# Autodesk Inventor assembly: EnsambleBaseMotor
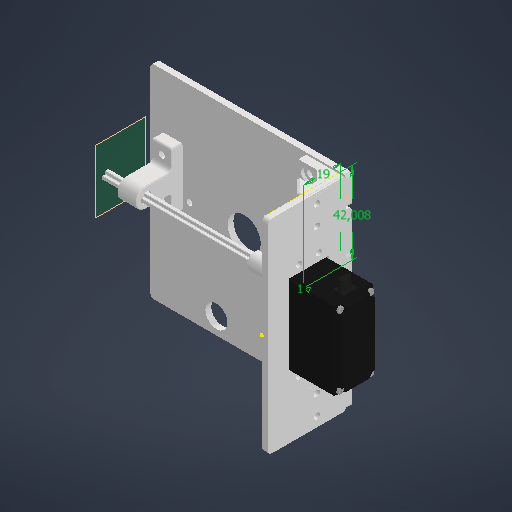
[picture p0: Inventor's stored thumbnail of the model, 512x512]
Saved by Autodesk Inventor 2026.3 (Build 303398000, 398)
## iProperties
Created: 2026-04-28
Part Number: EnsambleBaseMotor
Document SubType Name: Assembly
Designer: Jose Carlos
Author: Jose Carlos
## Documents named in this file (8)
- C:\Users\Caro\JoseCarlos\TEC\TFG\Inventor\PiezasSTD\EnsambleMotor\EnsambleBaseMotor.iam
- C:\Users\Caro\JoseCarlos\TEC\TFG\Inventor\PiezasSTD\EnsambleMotor\BaseMotoJose.ipt
- C:\Users\Caro\JoseCarlos\TEC\TFG\Inventor\PiezasSTD\EnsambleMotor\ParedEnsambleMotor.ipt
- C:\Users\Caro\JoseCarlos\TEC\TFG\Inventor\PiezasSTD\T.ipt
- C:\Users\Caro\JoseCarlos\TEC\TFG\Inventor\PiezasSTD\EnsambleMotor\AcopleMotor.ipt
- C:\Users\Caro\JoseCarlos\TEC\TFG\Inventor\PiezasSTD\EnsambleMotor\EjeDelMotor.ipt
- C:\Users\Caro\JoseCarlos\TEC\TFG\Inventor\Elementos\mg995-servo-motor-metal-gear-high-torque-standard-size-1.snapshot.1\MG995.ipt
- C:\Users\Caro\JoseCarlos\TEC\TFG\Inventor\PiezasSTD\EnsambleMotor\SoporteEjeMotor.ipt
## Components (12 placed, 7 different names)
1. BaseMotoJose:1 — Nivelación:1, Coincidencia:1, Coincidencia:4, Nivelación:3, Coincidencia:7, Nivelación:4, Coincidencia:9, Nivelación:5, Coincidencia:10, Ángulo:6, Nivelación:6, Ángulo:7, Coincidencia:26, Coincidencia:27, Coincidencia:28, Coincidencia:29, Coincidencia:30, Coincidencia:31, Ángulo:10, Ángulo:12
2. ParedEnsambleMotor:1 — Nivelación:1, Coincidencia:1, Ángulo:3, Coincidencia:5, Coincidencia:6, Coincidencia:22, Coincidencia:23, Ángulo:8, Ángulo:9
3. T:1 — Coincidencia:4, Ángulo:3, Coincidencia:5, Nivelación:3
4. T:2 — Coincidencia:6, Coincidencia:7, Nivelación:4
5. AcopleMotor:1 — Coincidencia:37, Coincidencia:38, Ángulo:12
6. EjeDelMotor:1 — Ángulo:6, Nivelación:8, Nivelación:9, Nivelación:10
7. MG995:1 — Coincidencia:22, Nivelación:6, Ángulo:7, Coincidencia:23, Ángulo:8, Ángulo:9
8. SoporteEjeMotor:1 — Nivelación:8, Nivelación:10
9. T:3 — Coincidencia:26, Coincidencia:27, Coincidencia:28, Ángulo:11, Coincidencia:32
10. T:4 — Coincidencia:29, Coincidencia:30, Coincidencia:31, Coincidencia:33
11. ParedEnsambleMotor:2 — Ángulo:10, Ángulo:11, Coincidencia:32, Coincidencia:33, Coincidencia:34, Coincidencia:35, Coincidencia:36
12. MG995:2 — Coincidencia:34, Coincidencia:35, Coincidencia:36, Coincidencia:37, Coincidencia:38, Nivelación:9
## Relationships (38: Mate 22, Flush 8, Angle 8)
- Nivelación:1 [Flush]: BaseMotoJose:1 ↔ ParedEnsambleMotor:1
- Coincidencia:1 [Mate]: BaseMotoJose:1 ↔ ParedEnsambleMotor:1
- Coincidencia:4 [Mate]: BaseMotoJose:1 ↔ T:1
- Ángulo:3 [Angle] (180 deg): ParedEnsambleMotor:1 ↔ T:1
- Coincidencia:5 [Mate]: ParedEnsambleMotor:1 ↔ T:1
- Nivelación:3 [Flush]: BaseMotoJose:1 ↔ T:1
- Coincidencia:6 [Mate]: ParedEnsambleMotor:1 ↔ T:2
- Coincidencia:7 [Mate]: BaseMotoJose:1 ↔ T:2
- Nivelación:4 [Flush]: BaseMotoJose:1 ↔ T:2
- Coincidencia:9 [Mate]: BaseMotoJose:1
- Nivelación:5 [Flush]: BaseMotoJose:1
- Coincidencia:10 [Mate]: BaseMotoJose:1
- Ángulo:6 [Angle] (0 deg): BaseMotoJose:1 ↔ EjeDelMotor:1
- Coincidencia:22 [Mate]: ParedEnsambleMotor:1 ↔ MG995:1
- Nivelación:6 [Flush]: BaseMotoJose:1 ↔ MG995:1
- Ángulo:7 [Angle] (0 deg): BaseMotoJose:1 ↔ MG995:1
- Coincidencia:23 [Mate]: ParedEnsambleMotor:1 ↔ MG995:1
- Ángulo:8 [Angle] (0 deg): ParedEnsambleMotor:1 ↔ MG995:1
- Ángulo:9 [Angle] (0 deg): ParedEnsambleMotor:1 ↔ MG995:1
- Nivelación:8 [Flush] (-10 mm): EjeDelMotor:1 ↔ SoporteEjeMotor:1
- Coincidencia:26 [Mate]: BaseMotoJose:1 ↔ T:3
- Coincidencia:27 [Mate]: BaseMotoJose:1 ↔ T:3
- Coincidencia:28 [Mate]: BaseMotoJose:1 ↔ T:3
- Coincidencia:29 [Mate]: BaseMotoJose:1 ↔ T:4
- Coincidencia:30 [Mate]: BaseMotoJose:1 ↔ T:4
- Coincidencia:31 [Mate]: BaseMotoJose:1 ↔ T:4
- Ángulo:10 [Angle] (180 deg): BaseMotoJose:1 ↔ ParedEnsambleMotor:2
- Ángulo:11 [Angle] (180 deg): T:3 ↔ ParedEnsambleMotor:2
- Coincidencia:32 [Mate]: T:3 ↔ ParedEnsambleMotor:2
- Coincidencia:33 [Mate]: T:4 ↔ ParedEnsambleMotor:2
- Coincidencia:34 [Mate]: ParedEnsambleMotor:2 ↔ MG995:2
- Coincidencia:35 [Mate]: ParedEnsambleMotor:2 ↔ MG995:2
- Coincidencia:36 [Mate]: ParedEnsambleMotor:2 ↔ MG995:2
- Coincidencia:37 [Mate]: AcopleMotor:1 ↔ MG995:2
- Coincidencia:38 [Mate]: AcopleMotor:1 ↔ MG995:2
- Ángulo:12 [Angle] (0 deg): BaseMotoJose:1 ↔ AcopleMotor:1
- Nivelación:9 [Flush]: EjeDelMotor:1 ↔ MG995:2
- Nivelación:10 [Flush] (10 mm): EjeDelMotor:1 ↔ SoporteEjeMotor:1
